# Autodesk Inventor assembly: Z Endstop-Unit
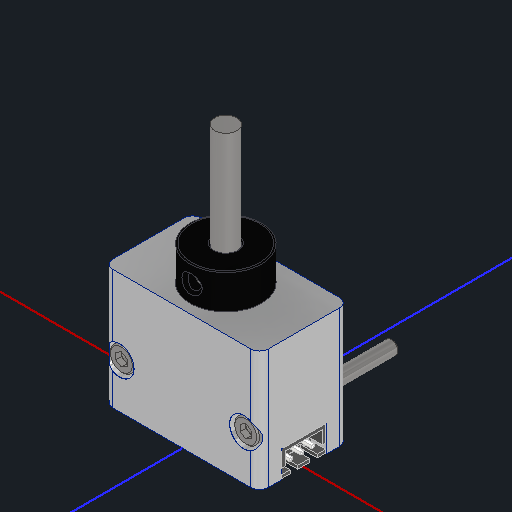
[picture p0: Inventor's stored thumbnail of the model, 512x512]
Saved by Autodesk Inventor 2022.2 (Build 262287010, 287A)
## iProperties
Created: 2022-03-17
Part Number: Z Endstop-Unit
Document SubType Name: Assembly
Designer: sleib
Author: sleib
## Documents named in this file (8)
- C:\Users\sleib\Projekte\Voron-2\CAD\Inventor\Z Endstop-Unit.iam
- C:\Users\sleib\Projekte\Voron-2\CAD\Inventor\Z Endstop v2.ipt
- Z Endstop.ipt
- C:\Users\sleib\Projekte\Voron-2\CAD\Inventor\JST XH 3 v3.ipt
- C:\Users\sleib\Projekte\Voron-2\CAD\Inventor\Microswitch Panasonic.ipt
- C:\Users\sleib\Projekte\Voron-2\CAD\Inventor\GT2 20T Pulley (6mm) Deflanged.ipt
- C:\Users\sleib\Projekte\Voron-2\CAD\Inventor\Pin 5x40.ipt
- C:\Users\sleib\Projekte\Voron-2\CAD\Inventor\M3x30 SHCS.ipt
## Components (7 placed, 6 different names)
1. Z Endstop:1 — Passend:1, Passend:2, Fluchtend:1, Passend:3, Passend:4, Passend:5, Tangential:1, Passend:6, Passend:7, Passend:10, Passend:11, Passend:12, Passend:13
2. JST XH 3 v3:1 — Passend:1, Passend:2, Fluchtend:1
3. Microswitch Panasonic:1 — Passend:3, Passend:4, Passend:5, Passend:9
4. GT2 20T Pulley (6mm) Deflanged:1 — Tangential:1, Passend:6, Passend:7, Passend:8
5. Pin 5x40:1 — Passend:8, Passend:9
6. M3x30 SHCS:1 — Passend:11, Passend:13
7. M3x30 SHCS:2 — Passend:10, Passend:12
## Relationships (15: Mate 13, Flush 1, Tangent 1)
- Passend:1 [Mate]: Z Endstop:1 ↔ JST XH 3 v3:1
- Passend:2 [Mate]: Z Endstop:1 ↔ JST XH 3 v3:1
- Fluchtend:1 [Flush]: Z Endstop:1 ↔ JST XH 3 v3:1
- Passend:3 [Mate]: Z Endstop:1 ↔ Microswitch Panasonic:1
- Passend:4 [Mate]: Z Endstop:1 ↔ Microswitch Panasonic:1
- Passend:5 [Mate]: Z Endstop:1 ↔ Microswitch Panasonic:1
- Tangential:1: Z Endstop:1 ↔ GT2 20T Pulley (6mm) Deflanged:1
- Passend:6 [Mate]: Z Endstop:1 ↔ GT2 20T Pulley (6mm) Deflanged:1
- Passend:7 [Mate]: Z Endstop:1 ↔ GT2 20T Pulley (6mm) Deflanged:1
- Passend:8 [Mate]: GT2 20T Pulley (6mm) Deflanged:1 ↔ Pin 5x40:1
- Passend:9 [Mate]: Microswitch Panasonic:1 ↔ Pin 5x40:1
- Passend:10 [Mate]: Z Endstop:1 ↔ M3x30 SHCS:2
- Passend:11 [Mate]: Z Endstop:1 ↔ M3x30 SHCS:1
- Passend:12 [Mate]: Z Endstop:1 ↔ M3x30 SHCS:2
- Passend:13 [Mate]: Z Endstop:1 ↔ M3x30 SHCS:1
